# Autodesk Inventor assembly: Full Assembly
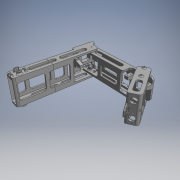
[picture p0: Inventor's stored thumbnail of the model, 180x180]
Saved by Autodesk Inventor 2020.5 (Build 245400000, 400)
## iProperties
Created: 2023-03-27
Part Number: Full Assembly
Document SubType Name: Assembly
Designer: Wes
Author: Wes
## Documents named in this file (4)
- C:\Users\Wes\Documents\Wes Stuff\Programming\Python\CPEN291\P2_L2B_G8\3D Design\Full Assembly.iam
- C:\Users\Wes\Documents\Wes Stuff\Programming\Python\CPEN291\P2_L2B_G8\3D Design\Arm Lower Shortened.iam
- C:\Users\Wes\Documents\Wes Stuff\Programming\Python\CPEN291\P2_L2B_G8\3D Design\Arm Middle.ipt
- C:\Users\Wes\Documents\Wes Stuff\Programming\Python\CPEN291\P2_L2B_G8\3D Design\Arm Upper.ipt
## Components (3 placed, 3 different names)
1. Arm Lower Shortened:1 [sub-assembly] — Rotational:1
2. Arm Middle:1 — Rotational:1, Rotational:2
3. Arm Upper:1 — Rotational:2
## Relationships (2: RevoluteJoint 2)
- Rotational:1 [RevoluteJoint]: Arm Lower Shortened:1 ↔ Arm Middle:1
- Rotational:2 [RevoluteJoint]: Arm Middle:1 ↔ Arm Upper:1
